# Autodesk Inventor assembly: BackTube
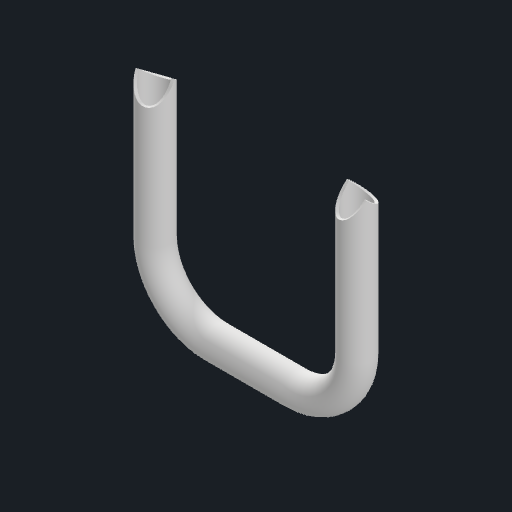
[picture p0: Inventor's stored thumbnail of the model, 512x512]
Saved by Autodesk Inventor 2025.2 (Build 292293000, 293)
## iProperties
Created: 2025-03-30
Part Number: BackTube
Document SubType Name: Assembly
Designer: valer
Author: valer
## Documents named in this file (2)
- C:\Users\valer\Desktop\str1ker\cad\BackTube.iam
- C:\Users\valer\Desktop\str1ker\cad\ChestBackTube.ipt
## Components (1 placed, 1 different names)
1. ChestBackTube:1 — Mate:1, Angle:1
## Relationships (2: Mate 1, Angle 1)
- Mate:1: ChestBackTube:1
- Angle:1 (0 deg): ChestBackTube:1
